# Autodesk Inventor assembly: PumpeV6
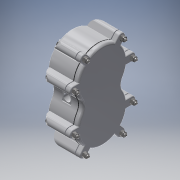
[picture p0: Inventor's stored thumbnail of the model, 180x180]
Saved by Autodesk Inventor 2017 (Build 210142000, 142)
## iProperties
Created: 2019-05-24
Part Number: PumpeV6
Document SubType Name: Assembly
Designer: Ole Simmering
Author: Ole Simmering
## Documents named in this file (8)
- C:\Users\Ole Simmering\Documents\3d modelling fun\HA4-Zahnradpumpe\PumpeV6.iam
- C:\Users\Ole Simmering\Documents\3d modelling fun\HA4-Zahnradpumpe\Gehaeuse_V6.ipt
- C:\Users\Ole Simmering\Documents\Inventor\Content Center Files\R2017\en-US\Bearing GB_T 292-2007\Rolling bearing B725 C GB_T 292-2007.ipt
- C:\Users\Ole Simmering\Documents\3d modelling fun\HA4-Zahnradpumpe\Zahnrad95x50.ipt
- C:\Users\Ole Simmering\Documents\Inventor\Content Center Files\R2017\en-US\ISO 4014(2)\ISO 4014 - M6 x 60 - ISO.ipt
- C:\Users\Ole Simmering\Documents\3d modelling fun\HA4-Zahnradpumpe\Dichtung.ipt
- C:\Users\Ole Simmering\Documents\3d modelling fun\HA4-Zahnradpumpe\Deckel.ipt
- C:\Users\Ole Simmering\Documents\Inventor\Content Center Files\R2017\en-US\DIN 986\DIN 986 - M6 x 1.ipt
## Components (25 placed, 7 different names)
1. Bearing GB/T 292-2007 Type IN - withdrawn B725 C:1 — Insert:3, Mate:3, Mate:4
2. Bearing GB/T 292-2007 Type IN - withdrawn B725 C:2 — Mate:1, Mate:2, Mate:5, Mate:6
3. Dichtung:1 — Mate:7, Mate:8, Mate:9
4. Bearing GB/T 292-2007 Type IN - withdrawn B725 C:3 — Mate:28, Mate:29
5. Bearing GB/T 292-2007 Type IN - withdrawn B725 C:4 — Mate:30, Mate:31
6. DIN 986 M6:1 — Mate:12, Mate:13
7. DIN 986 M6:2 — Mate:14, Mate:15
8. DIN 986 M6:3 — Mate:26, Mate:27
9. DIN 986 M6:4 — Mate:24, Mate:25
10. DIN 986 M6:5 — Mate:22, Mate:23
11. DIN 986 M6:6 — Mate:20, Mate:21
12. DIN 986 M6:7 — Mate:18, Mate:19
13. DIN 986 M6:8 — Mate:16, Mate:17
14. ISO 4014 M6 x 60:1 — Insert:10, Angle:2, Mate:12
15. ISO 4014 M6 x 60:2 — Insert:11, Angle:5, Mate:19
16. ISO 4014 M6 x 60:3 — Insert:9, Angle:3, Mate:15
17. ISO 4014 M6 x 60:4 — Insert:4, Angle:4, Mate:11, Mate:17
18. ISO 4014 M6 x 60:5 — Insert:5, Angle:1, Angle:6, Mate:21
19. ISO 4014 M6 x 60:6 — Insert:6, Angle:9, Mate:27
20. ISO 4014 M6 x 60:7 — Insert:7, Angle:8, Mate:10, Mate:25
21. ISO 4014 M6 x 60:8 — Insert:8, Angle:7, Mate:23
22. Gehaeuse_V6:1 — Insert:3, Mate:1, Mate:2, Insert:4, Insert:5, Insert:6, Insert:7, Insert:8, Insert:9, Insert:10, Insert:11, Angle:1, Angle:2, Angle:3, Angle:4, Angle:5, Angle:6, Angle:7, Angle:8, Angle:9, Mate:7, Mate:8
23. Zahnrad95x50:1 — Mate:3, Mate:4
24. Zahnrad95x50:2 — Mate:5, Mate:6
25. Deckel:1 — Mate:9, Mate:10, Mate:11, Mate:13, Mate:14, Mate:16, Mate:18, Mate:20, Mate:22, Mate:24, Mate:26, Mate:28, Mate:29, Mate:30, Mate:31
## Relationships (49: Mate 31, Insert 9, Angle 9)
- Insert:3: Bearing GB/T 292-2007 Type IN - withdrawn B725 C:1 ↔ Gehaeuse_V6:1
- Mate:1: Bearing GB/T 292-2007 Type IN - withdrawn B725 C:2 ↔ Gehaeuse_V6:1
- Mate:2: Bearing GB/T 292-2007 Type IN - withdrawn B725 C:2 ↔ Gehaeuse_V6:1
- Mate:3: Bearing GB/T 292-2007 Type IN - withdrawn B725 C:1 ↔ Zahnrad95x50:1
- Mate:4: Bearing GB/T 292-2007 Type IN - withdrawn B725 C:1 ↔ Zahnrad95x50:1
- Mate:5: Bearing GB/T 292-2007 Type IN - withdrawn B725 C:2 ↔ Zahnrad95x50:2
- Mate:6: Bearing GB/T 292-2007 Type IN - withdrawn B725 C:2 ↔ Zahnrad95x50:2
- Insert:4: ISO 4014 M6 x 60:4 ↔ Gehaeuse_V6:1
- Insert:5: ISO 4014 M6 x 60:5 ↔ Gehaeuse_V6:1
- Insert:6: ISO 4014 M6 x 60:6 ↔ Gehaeuse_V6:1
- Insert:7: ISO 4014 M6 x 60:7 ↔ Gehaeuse_V6:1
- Insert:8: ISO 4014 M6 x 60:8 ↔ Gehaeuse_V6:1
- Insert:9: ISO 4014 M6 x 60:3 ↔ Gehaeuse_V6:1
- Insert:10: ISO 4014 M6 x 60:1 ↔ Gehaeuse_V6:1
- Insert:11: ISO 4014 M6 x 60:2 ↔ Gehaeuse_V6:1
- Angle:1 (0 deg): ISO 4014 M6 x 60:5 ↔ Gehaeuse_V6:1
- Angle:2 (0 deg): ISO 4014 M6 x 60:1 ↔ Gehaeuse_V6:1
- Angle:3 (0 deg): ISO 4014 M6 x 60:3 ↔ Gehaeuse_V6:1
- Angle:4 (0 deg): ISO 4014 M6 x 60:4 ↔ Gehaeuse_V6:1
- Angle:5 (0 deg): ISO 4014 M6 x 60:2 ↔ Gehaeuse_V6:1
- Angle:6 (0 deg): ISO 4014 M6 x 60:5 ↔ Gehaeuse_V6:1
- Angle:7 (0 deg): ISO 4014 M6 x 60:8 ↔ Gehaeuse_V6:1
- Angle:8 (0 deg): ISO 4014 M6 x 60:7 ↔ Gehaeuse_V6:1
- Angle:9 (0 deg): ISO 4014 M6 x 60:6 ↔ Gehaeuse_V6:1
- Mate:7: Dichtung:1 ↔ Gehaeuse_V6:1
- Mate:8: Dichtung:1 ↔ Gehaeuse_V6:1
- Mate:9: Dichtung:1 ↔ Deckel:1
- Mate:10: ISO 4014 M6 x 60:7 ↔ Deckel:1
- Mate:11: ISO 4014 M6 x 60:4 ↔ Deckel:1
- Mate:12: DIN 986 M6:1 ↔ ISO 4014 M6 x 60:1
- Mate:13: DIN 986 M6:1 ↔ Deckel:1
- Mate:14: DIN 986 M6:2 ↔ Deckel:1
- Mate:15: DIN 986 M6:2 ↔ ISO 4014 M6 x 60:3
- Mate:16: DIN 986 M6:8 ↔ Deckel:1
- Mate:17: DIN 986 M6:8 ↔ ISO 4014 M6 x 60:4
- Mate:18: DIN 986 M6:7 ↔ Deckel:1
- Mate:19: DIN 986 M6:7 ↔ ISO 4014 M6 x 60:2
- Mate:20: DIN 986 M6:6 ↔ Deckel:1
- Mate:21: DIN 986 M6:6 ↔ ISO 4014 M6 x 60:5
- Mate:22: DIN 986 M6:5 ↔ Deckel:1
- Mate:23: DIN 986 M6:5 ↔ ISO 4014 M6 x 60:8
- Mate:24: DIN 986 M6:4 ↔ Deckel:1
- Mate:25: DIN 986 M6:4 ↔ ISO 4014 M6 x 60:7
- Mate:26: DIN 986 M6:3 ↔ Deckel:1
- Mate:27: DIN 986 M6:3 ↔ ISO 4014 M6 x 60:6
- Mate:28: Bearing GB/T 292-2007 Type IN - withdrawn B725 C:3 ↔ Deckel:1
- Mate:29: Bearing GB/T 292-2007 Type IN - withdrawn B725 C:3 ↔ Deckel:1
- Mate:30: Bearing GB/T 292-2007 Type IN - withdrawn B725 C:4 ↔ Deckel:1
- Mate:31: Bearing GB/T 292-2007 Type IN - withdrawn B725 C:4 ↔ Deckel:1
